# Autodesk Inventor assembly: 足首_独立ピッチ_1
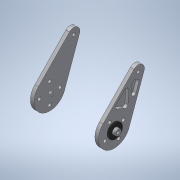
[picture p0: Inventor's stored thumbnail of the model, 180x180]
Saved by Autodesk Inventor 2020 (Build 240168000, 168)
## iProperties
Created: 2016-05-04
Part Number: 足首_独立ピッチ_1
Document SubType Name: Assembly
Designer: hiroaki
Mass: 12.4515 g
Surface Area: 78.9605 cm^2
Volume: 4.53639 cm^3
Density: 2.74481 g/cm^3
Author: hiroaki
## Documents named in this file (4)
- C:\Users\naoki\Documents\Inventor\CitBrains\git_clone\OpenPlatform167\足首再設計1\OpenPlatform_ver3_0\下半身\足首\足首_独立ピッチ_1.iam
- C:\Users\naoki\Documents\Inventor\CitBrains\git_clone\OpenPlatform167\足首再設計1\OpenPlatform_ver3_0\下半身\足首\足首_独立ピッチ_1_1.ipt
- C:\Users\naoki\Documents\Inventor\CitBrains\git_clone\OpenPlatform167\足首再設計1\OpenPlatform_ver3_0\既製品\CC-0512-10B.ipt
- C:\Users\naoki\Documents\Inventor\CitBrains\git_clone\OpenPlatform167\足首再設計1\OpenPlatform_ver3_0\既製品\新規購入\BRU-2604S.ipt
## Components (6 placed, 3 different names)
1. 足首_独立ピッチ_1_1:1 — メイト:2, メイト:5, メイト:6, 挿入:1
2. 足首_独立ピッチ_1_1:2 — メイト:2, メイト:6, 角度:1, 挿入:2
3. CC-0512-10B:1
4. CC-0512-10B:2
5. BRU-2604S:1 — 挿入:2
6. BRU-2604S:2 — 挿入:1
## Relationships (6: Mate 3, Insert 2, Angle 1)
- メイト:2 [Mate] (50.5 mm): 足首_独立ピッチ_1_1:1 ↔ 足首_独立ピッチ_1_1:2
- メイト:5 [Mate] (25.15 mm): 足首_独立ピッチ_1_1:1
- メイト:6 [Mate]: 足首_独立ピッチ_1_1:1 ↔ 足首_独立ピッチ_1_1:2
- 角度:1 [Angle] (0 deg): 足首_独立ピッチ_1_1:2
- 挿入:1 [Insert]: 足首_独立ピッチ_1_1:1 ↔ BRU-2604S:2
- 挿入:2 [Insert]: 足首_独立ピッチ_1_1:2 ↔ BRU-2604S:1
